# Autodesk Inventor assembly: GornjaKonstrukcija_v.1.1
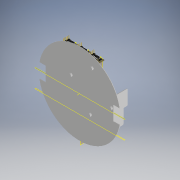
[picture p0: Inventor's stored thumbnail of the model, 180x180]
Saved by Autodesk Inventor 2020 (Build 240168000, 168)
## iProperties
Created: 2020-07-11
Part Number: GornjaKonstrukcija_v.1.1
Document SubType Name: Assembly
Designer: Sičaja
Author: Sičaja
## Documents named in this file (4)
- C:\Users\Sicaja\Documents\Draws_Inventor\Inventor_Robocup\GornjaKonstrukcija_v.1.1.iam
- C:\Users\Sicaja\Documents\Draws_Inventor\Inventor_Robocup\GonjaKonstrukcija_v.1.0.ipt
- C:\Users\Sicaja\Documents\Draws_Inventor\Inventor_Robocup\5DržačaLidara.ipt
- C:\Users\Sicaja\Documents\Draws_Inventor\Inventor_Robocup\mrm-lid-an.ipt
## Components (9 placed, 3 different names)
1. GonjaKonstrukcija_v.1.0:1 — Mate:1, Mate:4, Mate:5, Mate:6, Mate:7, Mate:8
2. 5DržačaLidara:1 — Mate:1, Mate:4, Mate:5, Mate:6, Mate:7, Insert:1, Insert:2, Insert:3, Insert:4, Insert:5, Insert:6
3. mrm-lid-an:3 — Insert:5, Insert:6
4. mrm-lid-an:2 — Insert:3, Insert:4
5. mrm-lid-an:1 — Insert:1, Insert:2
6. 5DržačaLidara:2
7. mrm-lid-an:4
8. mrm-lid-an:5
9. mrm-lid-an:6
## Component patterns: (2 elements, first: 5DržačaLidara:1 + mrm-lid-an:3 + mrm-lid-an:2 + mrm-lid-an:1)
## Relationships (12: Mate 6, Insert 6)
- Mate:1: GonjaKonstrukcija_v.1.0:1 ↔ 5DržačaLidara:1
- Mate:4: GonjaKonstrukcija_v.1.0:1 ↔ 5DržačaLidara:1
- Mate:5 (-3 mm): GonjaKonstrukcija_v.1.0:1 ↔ 5DržačaLidara:1
- Mate:6: GonjaKonstrukcija_v.1.0:1 ↔ 5DržačaLidara:1
- Mate:7: GonjaKonstrukcija_v.1.0:1 ↔ 5DržačaLidara:1
- Mate:8: GonjaKonstrukcija_v.1.0:1
- Insert:1: 5DržačaLidara:1 ↔ mrm-lid-an:1
- Insert:2: 5DržačaLidara:1 ↔ mrm-lid-an:1
- Insert:3: 5DržačaLidara:1 ↔ mrm-lid-an:2
- Insert:4: 5DržačaLidara:1 ↔ mrm-lid-an:2
- Insert:5: 5DržačaLidara:1 ↔ mrm-lid-an:3
- Insert:6: 5DržačaLidara:1 ↔ mrm-lid-an:3
